# Autodesk Inventor assembly: Main
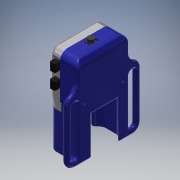
[picture p0: Inventor's stored thumbnail of the model, 180x180]
Saved by Autodesk Inventor 2018 (Build 220112000, 112)
## iProperties
Created: 2018-02-01
Part Number: Main
Document SubType Name: Assembly
Designer: Mandus
Author: Mandus
## Documents named in this file (9)
- C:\Users\Mandus\Dropbox\Skola\Projekt\Kretsn_Brillz_V2\3D\Main.iam
- C:\Users\Mandus\Dropbox\Skola\Projekt\Kretsn_Brillz_V2\3D\Powerbank.ipt
- C:\Users\Mandus\Dropbox\Skola\Projekt\Kretsn_Brillz_V2\3D\USB_Contact.ipt
- C:\Users\Mandus\Dropbox\Skola\Projekt\Kretsn_Brillz_V2\3D\Holster_Bottom.ipt
- C:\Users\Mandus\Dropbox\Skola\Projekt\Kretsn_Brillz_V2\3D\SchematicBKP_Shrinkwrap_1.ipt
- C:\Users\Mandus\Dropbox\Skola\Projekt\Kretsn_Brillz_V2\3D\Holster_Top.ipt
- C:\Users\Mandus\Dropbox\Skola\Projekt\Kretsn_Brillz_V2\3D\Holster_Button.ipt
- C:\Users\Mandus\Dropbox\Skola\Projekt\Kretsn_Brillz_V2\3D\Button_single.ipt
- C:\Users\Mandus\Dropbox\Skola\Projekt\Kretsn_Brillz_V2\3D\Holster_Top_V2.ipt
## Components (8 placed, 8 different names)
1. Powerbank:1 — Mate:1, Mate:2, Mate:3
2. USB_Contact:1 — Mate:1, Mate:2, Mate:3, Mate:4, Mate:5, Mate:7
3. Holster_Bottom:1 — Mate:4, Mate:5, Mate:6, Flush:2, Mate:7, Flush:3, Flush:4, Mate:9, Mate:19, Flush:6, Flush:7
4. SchematicBKP_Shrinkwrap_1:1 — Mate:6, Flush:2, Flush:3
5. Holster_Top:1 — Flush:4, Mate:9, Mate:19, Flush:6
6. Holster_Button:3 — Mate:20, Mate:21
7. Button_single:1 — Mate:22, Mate:23, Mate:24
8. Holster_Top_V2:1 — Flush:7, Mate:20, Mate:21, Mate:22, Mate:23, Mate:24
## Relationships (19: Mate 14, Flush 5)
- Mate:1: Powerbank:1 ↔ USB_Contact:1
- Mate:2 (0.3 mm): Powerbank:1 ↔ USB_Contact:1
- Mate:3: Powerbank:1 ↔ USB_Contact:1
- Mate:4: USB_Contact:1 ↔ Holster_Bottom:1
- Mate:5: USB_Contact:1 ↔ Holster_Bottom:1
- Mate:6: Holster_Bottom:1 ↔ SchematicBKP_Shrinkwrap_1:1
- Flush:2 (8.5 mm): Holster_Bottom:1 ↔ SchematicBKP_Shrinkwrap_1:1
- Mate:7: USB_Contact:1 ↔ Holster_Bottom:1
- Flush:3: Holster_Bottom:1 ↔ SchematicBKP_Shrinkwrap_1:1
- Flush:4: Holster_Bottom:1 ↔ Holster_Top:1
- Mate:9: Holster_Bottom:1 ↔ Holster_Top:1
- Mate:19: Holster_Bottom:1 ↔ Holster_Top:1
- Flush:6: Holster_Bottom:1 ↔ Holster_Top:1
- Flush:7: Holster_Bottom:1 ↔ Holster_Top_V2:1
- Mate:20: Holster_Button:3 ↔ Holster_Top_V2:1
- Mate:21 (0.5 mm): Holster_Button:3 ↔ Holster_Top_V2:1
- Mate:22: Button_single:1 ↔ Holster_Top_V2:1
- Mate:23 (0.5 mm): Button_single:1 ↔ Holster_Top_V2:1
- Mate:24 (0.7 mm): Button_single:1 ↔ Holster_Top_V2:1
